# Autodesk Inventor assembly: 17-0028-0019
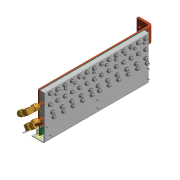
[picture p0: Inventor's stored thumbnail of the model, 180x180]
Saved by Autodesk Inventor 2016 SP2 (Build 200236200, 236)
## iProperties
Created: 2017-11-01
Part Number: 17-0028-0019
Document SubType Name: Assembly
Designer: Daan Giesen
Mass: 1921.85 g
Surface Area: 3089.59 cm^2
Volume: 451.015 cm^3
Density: 4.26118 g/cm^3
Project: Digital PID Loop
Cost Center: 17-0028
User Status: CNC
Authority: Reichsöllner, Lukas
RuleStatus: InUse
Category: -
Company: Universiteit van Amsterdam
BeforeDocSave0: Show Form
Author: Daan Giesen
Title: Digital PID Loop
Revision Number: A.1
## Documents named in this file (20)
- D:\VaultLocalWorkingFolder\UvA_MT\Projects\2017\17-0028 Digital PID Loop\10_Assemblies\17-0028-0019.iam
- D:\VaultLocalWorkingFolder\UvA_MT\Projects\2017\17-0028 Digital PID Loop\20_3D-Models\17-0028-0016.ipt
- D:\VaultLocalWorkingFolder\UvA_MT\Projects\2017\17-0028 Digital PID Loop\20_3D-Models\17-0028-0017.ipt
- D:\VaultLocalWorkingFolder\UvA_MT\Projects\2017\17-0028 Digital PID Loop\20_3D-Models\17-0028-0018.ipt
- D:\VaultLocalWorkingFolder\UvA_MT\Projects\2017\17-0028 Digital PID Loop\20_3D-Models\hsa5r10j.ipt
- D:\VaultLocalWorkingFolder\UvA_MT\Projects\2017\17-0028 Digital PID Loop\20_3D-Models\17-0028-0022.ipt
- D:\VaultLocalWorkingFolder\UvA_MT\Projects\2017\17-0028 Digital PID Loop\20_3D-Models\17-0028-0024.ipt
- \\home.uva.nl\dgiesen1\Inventor\Content Center Files\R2016\en-US\DIN EN ISO 7089\DIN EN ISO 7089 -  3.ipt
- \\home.uva.nl\dgiesen1\Inventor\Content Center Files\R2016\en-US\DIN EN ISO 4032\DIN EN ISO 4032 - M3.ipt
- D:\VaultLocalWorkingFolder\UvA_MT\Projects\2017\17-0028 Digital PID Loop\20_3D-Models\17-0028-0026.ipt
- \\home.uva.nl\dgiesen1\Inventor\Content Center Files\R2016\en-US\ISO 4762(1)\DIN EN ISO 4762 - M4 x 20.ipt
- D:\VaultLocalWorkingFolder\UvA_MT\Projects\2017\17-0028 Digital PID Loop\20_3D-Models\17-0028-0027.ipt
- D:\VaultLocalWorkingFolder\UvA_MT\Projects\2017\17-0028 Digital PID Loop\20_3D-Models\17-0028-0031.ipt
- D:\VaultLocalWorkingFolder\UvA_MT\Projects\2017\17-0028 Digital PID Loop\20_3D-Models\17-0028-0096.iam
- D:\VaultLocalWorkingFolder\UvA_MT\Projects\2017\17-0028 Digital PID Loop\20_3D-Models\B-6M0-9-SwagelokCompany-12-13-2017.ipt
- D:\VaultLocalWorkingFolder\UvA_MT\Projects\2017\17-0028 Digital PID Loop\20_3D-Models\17-0028-0104.ipt
- D:\VaultLocalWorkingFolder\UvA_MT\Projects\2017\17-0028 Digital PID Loop\20_3D-Models\17-0028-0105.ipt
- \\home.uva.nl\dgiesen1\Inventor\Content Center Files\R2016\en-US\ISO 4762(1)\DIN EN ISO 4762 - M2 x 6.ipt
- D:\VaultLocalWorkingFolder\UvA_MT\Projects\2017\17-0028 Digital PID Loop\20_3D-Models\17-0028-0118.ipt
- \\home.uva.nl\dgiesen1\Inventor\Content Center Files\R2016\en-US\ISO 4762(1)\DIN EN ISO 4762 - M3 x 30.ipt
## Components (200 placed, 19 different names)
1. 17-0028-0016:1 — Flush:1, Flush:2, Flush:4, Mate:17, Flush:7, Flush:8, Flush:9, Mate:50, Mate:52, Mate:62, Mate:70, Flush:12, Mate:82
2. 17-0028-0017:1 — Flush:1, Flush:4, Mate:49, Mate:74, Mate:79, Mate:91
3. 17-0028-0018:1 — Flush:2, Mate:19, Flush:9, Angle:1, Flush:11, Mate:80, Mate:89, Mate:90
4. 17-0028-0022:1 — Mate:50, Mate:52, Mate:82, Mate:83, Mate:84, Mate:85, Mate:86
5. 17-0028-0024:1 — Mate:17, Flush:7, Flush:8, Mate:48, Mate:57, Mate:58, Mate:61, Mate:66, Mate:69, Mate:73, Mate:81
6. 17-0028-0027:1 — Flush:12, Mate:79, Mate:80
7. 17-0028-0096:1 [sub-assembly]
8. B-6M0-9-SwagelokCompany-12-13-2017:1 — Mate:83, Mate:86, Angle:2
9. B-6M0-9-SwagelokCompany-12-13-2017:2 — Mate:84, Mate:85, Mate:87, Mate:88, Angle:2
10. 17-0028-0104:1 — Mate:87, Mate:88
11. DIN EN ISO 4762 M4 x 20:1 — Mate:46, Mate:47
12. 17-0028-0026:1 — Mate:46, Mate:47, Mate:48, Mate:49
13. DIN EN ISO 4762 M4 x 20:3
14. 17-0028-0026:3
15. DIN EN ISO 4762 M4 x 20:4
16. 17-0028-0026:4
17. DIN EN ISO 4762 M4 x 20:5
18. 17-0028-0026:5
19. DIN EN ISO 4762 M4 x 20:6
20. 17-0028-0026:6
21. DIN EN ISO 4762 M4 x 20:7
22. 17-0028-0026:7
23. DIN EN ISO 4762 M4 x 20:8
24. 17-0028-0026:8
25. DIN EN ISO 4762 M4 x 20:9
26. 17-0028-0026:9
27. DIN EN ISO 4762 M4 x 20:10
28. 17-0028-0026:10
29. DIN EN ISO 4762 M4 x 20:11
30. 17-0028-0026:11
31. DIN EN ISO 4762 M4 x 20:12
32. 17-0028-0026:12
33. DIN EN ISO 4762 M4 x 20:13
34. 17-0028-0026:13
35. DIN EN ISO 4762 M4 x 20:14
36. 17-0028-0026:14
37. DIN EN ISO 4762 M4 x 20:15
38. 17-0028-0026:15
39. DIN EN ISO 4762 M4 x 20:16
40. 17-0028-0026:16
41. DIN EN ISO 4762 M4 x 20:17
42. 17-0028-0026:17
43. DIN EN ISO 4762 M4 x 20:18
44. 17-0028-0026:18
45. DIN EN ISO 4762 M4 x 20:19
46. 17-0028-0026:19
47. DIN EN ISO 4762 M4 x 20:20
48. 17-0028-0026:20
49. DIN EN ISO 4762 M4 x 20:21
50. 17-0028-0026:21
51. DIN EN ISO 4762 M4 x 20:22
52. 17-0028-0026:22
53. DIN EN ISO 4762 M4 x 20:23
54. 17-0028-0026:23
55. DIN EN ISO 4762 M4 x 20:24
56. 17-0028-0026:24
57. DIN EN ISO 4762 M4 x 20:25
58. 17-0028-0026:25
59. DIN EN ISO 4762 M4 x 20:26
60. 17-0028-0026:26
61. DIN EN ISO 4762 M4 x 20:27
62. 17-0028-0026:27
63. DIN EN ISO 4762 M4 x 20:28
64. 17-0028-0026:28
65. DIN EN ISO 4762 M4 x 20:29
66. 17-0028-0026:29
67. DIN EN ISO 4762 M4 x 20:30
68. 17-0028-0026:30 — Mate:61, Mate:62
69. 17-0028-0026:2 — Mate:57
70. DIN EN ISO 4762 M4 x 20:2 — Mate:58
71. DIN EN ISO 4762 M4 x 20:31
72. 17-0028-0026:31
73. 17-0028-0026:32
74. DIN EN ISO 4762 M4 x 20:32
75. DIN EN ISO 4762 M4 x 20:33
76. 17-0028-0026:33
77. 17-0028-0026:34
78. DIN EN ISO 4762 M4 x 20:34
79. DIN EN ISO 4762 M4 x 20:35
80. 17-0028-0026:35
81. 17-0028-0026:36
82. DIN EN ISO 4762 M4 x 20:36
83. DIN EN ISO 4762 M4 x 20:37
84. 17-0028-0026:37
85. 17-0028-0026:38
86. DIN EN ISO 4762 M4 x 20:38
87. DIN EN ISO 4762 M4 x 20:39
88. 17-0028-0026:39
89. 17-0028-0026:40
90. DIN EN ISO 4762 M4 x 20:40
91. DIN EN ISO 4762 M4 x 20:41
92. 17-0028-0026:41 — Mate:66, Mate:81
93. DIN EN ISO 4762 M4 x 20:42
94. 17-0028-0026:42 — Mate:69, Mate:70
95. DIN EN ISO 4762 M4 x 20:43
96. 17-0028-0026:43
97. DIN EN ISO 4762 M4 x 20:44
98. 17-0028-0026:44
99. DIN EN ISO 4762 M4 x 20:45
100. 17-0028-0026:45
101. DIN EN ISO 4762 M4 x 20:46
102. 17-0028-0026:46
103. DIN EN ISO 4762 M4 x 20:47
104. 17-0028-0026:47
105. DIN EN ISO 4762 M4 x 20:48
106. 17-0028-0026:48
107. DIN EN ISO 4762 M4 x 20:49
108. 17-0028-0026:49
109. DIN EN ISO 4762 M4 x 20:50
110. 17-0028-0026:50
111. DIN EN ISO 4762 M3 x 30:1 — Insert:50, Mate:75, Mate:77, Mate:92
112. DIN EN ISO 4032 M3:3 — Mate:77, Mate:78
113. DIN EN ISO 7089 3:1 — Mate:75, Mate:78
114. 17-0028-0118:1 — Mate:91, Mate:92
115. hsa5r10j:1 — Mate:19, Angle:1, Flush:11, Insert:22, Insert:24
116. DIN EN ISO 4762 M2 x 6:1 — Insert:22
117. DIN EN ISO 4762 M2 x 6:21 — Insert:24
118. 17-0028-0031:1 — Mate:73, Mate:74, Insert:50
119. 17-0028-0105:1 — Mate:89, Mate:90
120. DIN EN ISO 4762 M3 x 30:2
121. DIN EN ISO 4032 M3:4
122. DIN EN ISO 7089 3:2
123. 17-0028-0118:2
124. hsa5r10j:2
125. DIN EN ISO 4762 M2 x 6:22
126. DIN EN ISO 4762 M2 x 6:23
127. 17-0028-0031:2
128. 17-0028-0105:2
129. DIN EN ISO 4762 M3 x 30:3
130. DIN EN ISO 4032 M3:5
131. DIN EN ISO 7089 3:3
132. 17-0028-0118:3
133. hsa5r10j:3
134. DIN EN ISO 4762 M2 x 6:24
135. DIN EN ISO 4762 M2 x 6:25
136. 17-0028-0031:3
137. 17-0028-0105:3
138. DIN EN ISO 4762 M3 x 30:4
139. DIN EN ISO 4032 M3:6
140. DIN EN ISO 7089 3:4
141. 17-0028-0118:4
142. hsa5r10j:4
143. DIN EN ISO 4762 M2 x 6:26
144. DIN EN ISO 4762 M2 x 6:27
145. 17-0028-0031:4
146. 17-0028-0105:4
147. DIN EN ISO 4762 M3 x 30:5
148. DIN EN ISO 4032 M3:7
149. DIN EN ISO 7089 3:5
150. 17-0028-0118:5
151. hsa5r10j:5
152. DIN EN ISO 4762 M2 x 6:28
153. DIN EN ISO 4762 M2 x 6:29
154. 17-0028-0031:5
155. 17-0028-0105:5
156. DIN EN ISO 4762 M3 x 30:6
157. DIN EN ISO 4032 M3:8
158. DIN EN ISO 7089 3:6
159. 17-0028-0118:6
160. hsa5r10j:6
161. DIN EN ISO 4762 M2 x 6:30
162. DIN EN ISO 4762 M2 x 6:31
163. 17-0028-0031:6
164. 17-0028-0105:6
165. DIN EN ISO 4762 M3 x 30:7
166. DIN EN ISO 4032 M3:9
167. DIN EN ISO 7089 3:7
168. 17-0028-0118:7
169. hsa5r10j:7
170. DIN EN ISO 4762 M2 x 6:32
171. DIN EN ISO 4762 M2 x 6:33
172. 17-0028-0031:7
173. 17-0028-0105:7
174. DIN EN ISO 4762 M3 x 30:8
175. DIN EN ISO 4032 M3:10
176. DIN EN ISO 7089 3:8
177. 17-0028-0118:8
178. hsa5r10j:8
179. DIN EN ISO 4762 M2 x 6:34
180. DIN EN ISO 4762 M2 x 6:35
181. 17-0028-0031:8
182. 17-0028-0105:8
183. DIN EN ISO 4762 M3 x 30:9
184. DIN EN ISO 4032 M3:11
185. DIN EN ISO 7089 3:9
186. 17-0028-0118:9
187. hsa5r10j:9
188. DIN EN ISO 4762 M2 x 6:36
189. DIN EN ISO 4762 M2 x 6:37
190. 17-0028-0031:9
191. 17-0028-0105:9
192. DIN EN ISO 4762 M3 x 30:10
193. DIN EN ISO 4032 M3:12
194. DIN EN ISO 7089 3:10
195. 17-0028-0118:10
196. hsa5r10j:10
197. DIN EN ISO 4762 M2 x 6:38
198. DIN EN ISO 4762 M2 x 6:39
199. 17-0028-0031:10
200. 17-0028-0105:10
## Component patterns: (28 elements, first: DIN EN ISO 4762 M4 x 20:1 + 17-0028-0026:1), (6 elements, first: DIN EN ISO 4762 M4 x 20:30 + 17-0028-0026:30 + 17-0028-0026:2 + DIN EN ISO 4762 M4 x 20:2), (5 elements, first: DIN EN ISO 4762 M4 x 20:41 + 17-0028-0026:41 + DIN EN ISO 4762 M4 x 20:42 + 17-0028-0026:42), (2 elements), (5 elements, first: DIN EN ISO 4762 M3 x 30:1 + DIN EN ISO 4032 M3:3 + DIN EN ISO 7089 3:1 + 17-0028-0118:1 + hsa5r10j:1 + DIN EN ISO 4762 M2 x 6:1 + DIN EN ISO 4762 M2 x 6:21 + 17-0028-0031:1 + 17-0028-0105:1), Component Pattern 12:2 (5 elements)
## Relationships (58: Mate 44, Flush 9, Insert 3, Angle 2)
- Flush:1: 17-0028-0016:1 ↔ 17-0028-0017:1
- Flush:2: 17-0028-0016:1 ↔ 17-0028-0018:1
- Flush:4: 17-0028-0016:1 ↔ 17-0028-0017:1
- Mate:17: 17-0028-0016:1 ↔ 17-0028-0024:1
- Flush:7: 17-0028-0016:1 ↔ 17-0028-0024:1
- Flush:8: 17-0028-0016:1 ↔ 17-0028-0024:1
- Mate:19: 17-0028-0018:1 ↔ hsa5r10j:1
- [Mate]: 17-0028-0024:1 ↔ 17-0028-0096:1
- [Mate] (8 mm): 17-0028-0024:1 ↔ 17-0028-0096:1
- Flush:9: 17-0028-0016:1 ↔ 17-0028-0018:1
- Angle:1 (0 deg): 17-0028-0018:1 ↔ hsa5r10j:1
- [Flush]: 17-0028-0024:1 ↔ 17-0028-0096:1
- Flush:11 (2 mm): 17-0028-0018:1 ↔ hsa5r10j:1
- Mate:46: DIN EN ISO 4762 M4 x 20:1 ↔ 17-0028-0026:1
- Mate:47: DIN EN ISO 4762 M4 x 20:1 ↔ 17-0028-0026:1
- Mate:48: 17-0028-0024:1 ↔ 17-0028-0026:1
- Mate:49: 17-0028-0017:1 ↔ 17-0028-0026:1
- Mate:50: 17-0028-0016:1 ↔ 17-0028-0022:1
- Mate:52: 17-0028-0016:1 ↔ 17-0028-0022:1
- Insert:22: hsa5r10j:1 ↔ DIN EN ISO 4762 M2 x 6:1
- Insert:24: hsa5r10j:1 ↔ DIN EN ISO 4762 M2 x 6:21
- [Mate]: 17-0028-0026:2 ↔ DIN EN ISO 4762 M4 x 20:2
- [Mate]: 17-0028-0026:2 ↔ DIN EN ISO 4762 M4 x 20:2
- Mate:57: 17-0028-0024:1 ↔ 17-0028-0026:2
- Mate:58: 17-0028-0024:1 ↔ DIN EN ISO 4762 M4 x 20:2
- [Mate]: DIN EN ISO 4762 M4 x 20:30 ↔ 17-0028-0026:30
- [Mate]: DIN EN ISO 4762 M4 x 20:30 ↔ 17-0028-0026:30
- Mate:61: 17-0028-0024:1 ↔ 17-0028-0026:30
- Mate:62: 17-0028-0016:1 ↔ 17-0028-0026:30
- [Mate]: DIN EN ISO 4762 M4 x 20:41 ↔ 17-0028-0026:41
- [Mate]: DIN EN ISO 4762 M4 x 20:41 ↔ 17-0028-0026:41
- Mate:66: 17-0028-0024:1 ↔ 17-0028-0026:41
- [Mate]: DIN EN ISO 4762 M4 x 20:42 ↔ 17-0028-0026:42
- [Mate]: DIN EN ISO 4762 M4 x 20:42 ↔ 17-0028-0026:42
- Mate:69: 17-0028-0024:1 ↔ 17-0028-0026:42
- Mate:70: 17-0028-0016:1 ↔ 17-0028-0026:42
- Flush:12: 17-0028-0016:1 ↔ 17-0028-0027:1
- Mate:73: 17-0028-0024:1 ↔ 17-0028-0031:1
- Mate:74: 17-0028-0017:1 ↔ 17-0028-0031:1
- Insert:50: DIN EN ISO 4762 M3 x 30:1 ↔ 17-0028-0031:1
- Mate:75: DIN EN ISO 4762 M3 x 30:1 ↔ DIN EN ISO 7089 3:1
- Mate:77: DIN EN ISO 4762 M3 x 30:1 ↔ DIN EN ISO 4032 M3:3
- Mate:78: DIN EN ISO 4032 M3:3 ↔ DIN EN ISO 7089 3:1
- Mate:79: 17-0028-0017:1 ↔ 17-0028-0027:1
- Mate:80: 17-0028-0018:1 ↔ 17-0028-0027:1
- Mate:81: 17-0028-0024:1 ↔ 17-0028-0026:41
- Mate:82: 17-0028-0016:1 ↔ 17-0028-0022:1
- Mate:83: 17-0028-0022:1 ↔ B-6M0-9-SwagelokCompany-12-13-2017:1
- Mate:84: 17-0028-0022:1 ↔ B-6M0-9-SwagelokCompany-12-13-2017:2
- Mate:85: 17-0028-0022:1 ↔ B-6M0-9-SwagelokCompany-12-13-2017:2
- Mate:86: 17-0028-0022:1 ↔ B-6M0-9-SwagelokCompany-12-13-2017:1
- Mate:87: B-6M0-9-SwagelokCompany-12-13-2017:2 ↔ 17-0028-0104:1
- Mate:88: B-6M0-9-SwagelokCompany-12-13-2017:2 ↔ 17-0028-0104:1
- Angle:2 (180 deg): B-6M0-9-SwagelokCompany-12-13-2017:1 ↔ B-6M0-9-SwagelokCompany-12-13-2017:2
- Mate:89: 17-0028-0018:1 ↔ 17-0028-0105:1
- Mate:90: 17-0028-0018:1 ↔ 17-0028-0105:1
- Mate:91: 17-0028-0017:1 ↔ 17-0028-0118:1
- Mate:92: DIN EN ISO 4762 M3 x 30:1 ↔ 17-0028-0118:1
## Named parameters: n_array = 5, d_array = 26 mm, D_pipe = 1 mm, d129_d106 = 0 mm, d130_d107 = 0 mm, d137_d129_d106 = 0 mm, d138_d130_d107 = 0 mm, d145_d129_d106 = 0 mm, d146_d130_d107 = 0 mm, d149_d129_d106 = 0 mm, d150_d130_d107 = 0 mm
